# Autodesk Inventor assembly: 4_Bar_Linkage
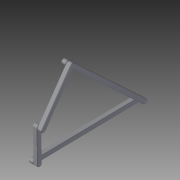
[picture p0: Inventor's stored thumbnail of the model, 180x180]
Saved by Autodesk Inventor 2015 (Build 190159000, 159)
## iProperties
Created: 2015-04-08
Part Number: 4_Bar_Linkage
Document SubType Name: Assembly
Designer: WASHHSST
Author: WASHHSST
## Documents named in this file (5)
- C:\Users\washhsst\Documents\GitHub\myWork\4_Bar_Linkage\4_Bar_Linkage.iam
- C:\Users\washhsst\Documents\GitHub\myWork\4_Bar_Linkage\bar.ipt
- C:\Users\washhsst\Documents\GitHub\myWork\4_Bar_Linkage\pin.ipt
- C:\Users\washhsst\Documents\GitHub\myWork\4_Bar_Linkage\longerBar.ipt
- C:\Users\washhsst\Documents\GitHub\myWork\4_Bar_Linkage\shortBar.ipt
## Components (8 placed, 4 different names)
1. bar:1 — Insert:5, Insert:9, Angle:1
2. pin:1 — Insert:5, Insert:10
3. pin:2 — Insert:11, Insert:12
4. pin:3 — Insert:13, Mate:1
5. bar:4 — Insert:8, Insert:11
6. pin:4 — Insert:8, Insert:9
7. longerBar:1 — Insert:12, Mate:1
8. shortBar:1 — Insert:10, Insert:13, Angle:1
## Relationships (9: Insert 7, Mate 1, Angle 1)
- Insert:5: bar:1 ↔ pin:1
- Insert:8: bar:4 ↔ pin:4
- Insert:9: bar:1 ↔ pin:4
- Insert:10: pin:1 ↔ shortBar:1
- Insert:11: pin:2 ↔ bar:4
- Insert:12: pin:2 ↔ longerBar:1
- Insert:13: pin:3 ↔ shortBar:1
- Mate:1: pin:3 ↔ longerBar:1
- Angle:1 (90 deg): bar:1 ↔ shortBar:1
